# Autodesk Inventor assembly: WheelAndFlywheel
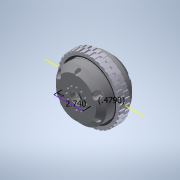
[picture p0: Inventor's stored thumbnail of the model, 180x180]
Saved by Autodesk Inventor 2020 (Build 240168000, 168)
## iProperties
Created: 2017-12-13
Part Number: WheelAndFlywheel
Document SubType Name: Assembly
Designer: Autodesk Inc.
Catalog Web Link: http://www.andymark.com/product-p/am-0940.htm
Vendor: AndyMark Inc.
Mass: 226.796 g
Surface Area: 1150.49 cm^2
Volume: 196.611 cm^3
Category: Loose Items
Company: Autodesk Inc.
Author: Autodesk Inc.
Keywords: Drive Base Kit
## Documents named in this file (6)
- C:\Users\srini\Documents\FRC\2020\Shooter\WheelAndFlywheel.iam
- C:\Users\srini\Documents\FRC\2020\2018_KOP\Inventor\FRC 2018 Drive Base Kit Inventor\FIRST 2018 Drive Base Kit\Parts\6 HiGrip Tread.ipt
- C:\Users\srini\Documents\FRC\2020\2018_KOP\Inventor\FRC 2018 Drive Base Kit Inventor\FIRST 2018 Drive Base Kit\Parts\6in 2008 FIRST Hub.ipt
- C:\Users\srini\Documents\FRC\2020\Shooter\Flywheel.ipt
- C:\Users\srini\Documents\FRC\2020\Shooter\BottomInsert_A.ipt
- C:\Users\srini\Documents\FRC\2020\Shooter\TopFlywheelClamp.ipt
## Components (8 placed, 5 different names)
1. 6 HiGrip Tread:1 — Mate:4, Flush:2
2. 6in 2008 FIRST Hub:1 — Mate:1, Mate:2, Mate:3, Angle:1, Flush:1, Mate:4, Flush:2, Mate:7, Mate:8
3. Flywheel:1 — Mate:1, Mate:5, Insert:1
4. Flywheel:2 — Mate:2, Mate:9, Insert:2
5. BottomInsert_A:1 — Flush:3, Mate:5, Mate:6
6. BottomInsert_A:2 — Mate:6, Mate:7, Mate:8, Mate:9
7. TopFlywheelClamp:1 — Insert:1
8. TopFlywheelClamp:2 — Insert:2
## Relationships (15: Mate 9, Flush 3, Insert 2, Angle 1)
- Mate:1: 6in 2008 FIRST Hub:1 ↔ Flywheel:1
- Mate:2: 6in 2008 FIRST Hub:1 ↔ Flywheel:2
- Mate:3: 6in 2008 FIRST Hub:1
- Angle:1 (0 deg): 6in 2008 FIRST Hub:1
- Flush:1 (-1.5748 mm): 6in 2008 FIRST Hub:1
- Mate:4: 6 HiGrip Tread:1 ↔ 6in 2008 FIRST Hub:1
- Flush:2: 6 HiGrip Tread:1 ↔ 6in 2008 FIRST Hub:1
- Flush:3: BottomInsert_A:1
- Mate:5: Flywheel:1 ↔ BottomInsert_A:1
- Mate:6: BottomInsert_A:1 ↔ BottomInsert_A:2
- Mate:7: 6in 2008 FIRST Hub:1 ↔ BottomInsert_A:2
- Mate:8: 6in 2008 FIRST Hub:1 ↔ BottomInsert_A:2
- Mate:9: Flywheel:2 ↔ BottomInsert_A:2
- Insert:1: Flywheel:1 ↔ TopFlywheelClamp:1
- Insert:2: Flywheel:2 ↔ TopFlywheelClamp:2
